# Autodesk Inventor assembly: base_assem
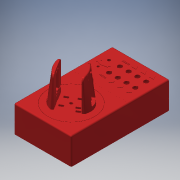
[picture p0: Inventor's stored thumbnail of the model, 180x180]
Saved by Autodesk Inventor 2018.2 (Build 222227000, 227)
## iProperties
Created: 2014-04-22
Part Number: base_assem
Document SubType Name: Assembly
Designer: t_emanb
Author: t_emanb
## Documents named in this file (9)
- C:\Users\mcnameed\git\carrickdojo\3D Printing\RoboticArm\base_assem.iam
- C:\Users\mcnameed\git\carrickdojo\3D Printing\RoboticArm\base_bottombuttonsBox.ipt
- C:\Users\mcnameed\git\carrickdojo\3D Printing\RoboticArm\base_bottomrotateBox.ipt
- C:\Users\mcnameed\git\carrickdojo\3D Printing\RoboticArm\base_topbuttonsBox.ipt
- C:\Users\mcnameed\git\carrickdojo\3D Printing\RoboticArm\base_toprotateBox.ipt
- C:\Users\mcnameed\git\carrickdojo\3D Printing\RoboticArm\base_bottomrotate.ipt
- C:\Users\mcnameed\git\carrickdojo\3D Printing\RoboticArm\base_toprotate.ipt
- C:\Users\mcnameed\git\carrickdojo\3D Printing\RoboticArm\base_servomountcurve.ipt
- C:\Users\mcnameed\git\carrickdojo\3D Printing\RoboticArm\base_servomountcurveMirror.ipt
## Components (8 placed, 8 different names)
1. base_bottombuttonsBox:1 — Flush:1, Mate:1, Flush:2, Flush:7, Mate:2
2. base_bottomrotateBox:1 — Flush:1, Mate:1, Flush:2, Flush:5, Flush:6
3. base_topbuttonsBox:1 — Flush:3, Flush:4, Flush:5, Flush:6
4. base_toprotateBox:1 — Flush:3, Flush:4, Flush:7, Mate:2, Flush:8, Mate:49
5. base_bottomrotate:1 — Mate:5, Mate:50, Mate:51
6. base_toprotate:1 — Mate:5, Flush:8, Mate:41, Mate:42, Mate:43, Mate:44, Mate:45, Mate:46, Mate:49, Mate:50, Mate:51
7. base_servomountcurve:1 — Mate:41, Mate:42, Mate:43
8. base_servomountcurveMirror:1 — Mate:44, Mate:45, Mate:46
## Relationships (20: Mate 12, Flush 8)
- Flush:1: base_bottombuttonsBox:1 ↔ base_bottomrotateBox:1
- Mate:1: base_bottombuttonsBox:1 ↔ base_bottomrotateBox:1
- Flush:2: base_bottombuttonsBox:1 ↔ base_bottomrotateBox:1
- Flush:3: base_topbuttonsBox:1 ↔ base_toprotateBox:1
- Flush:4: base_topbuttonsBox:1 ↔ base_toprotateBox:1
- Flush:5: base_bottomrotateBox:1 ↔ base_topbuttonsBox:1
- Flush:6: base_bottomrotateBox:1 ↔ base_topbuttonsBox:1
- Flush:7: base_bottombuttonsBox:1 ↔ base_toprotateBox:1
- Mate:2: base_bottombuttonsBox:1 ↔ base_toprotateBox:1
- Mate:5: base_bottomrotate:1 ↔ base_toprotate:1
- Flush:8: base_toprotateBox:1 ↔ base_toprotate:1
- Mate:41: base_toprotate:1 ↔ base_servomountcurve:1
- Mate:42: base_toprotate:1 ↔ base_servomountcurve:1
- Mate:43: base_toprotate:1 ↔ base_servomountcurve:1
- Mate:44: base_toprotate:1 ↔ base_servomountcurveMirror:1
- Mate:45: base_toprotate:1 ↔ base_servomountcurveMirror:1
- Mate:46: base_toprotate:1 ↔ base_servomountcurveMirror:1
- Mate:49: base_toprotateBox:1 ↔ base_toprotate:1
- Mate:50: base_bottomrotate:1 ↔ base_toprotate:1
- Mate:51: base_bottomrotate:1 ↔ base_toprotate:1
